# Autodesk Inventor assembly: 5_left_Arm
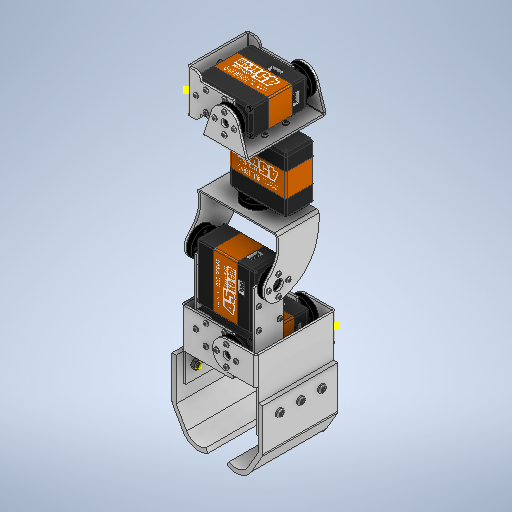
[picture p0: Inventor's stored thumbnail of the model, 512x512]
Saved by Autodesk Inventor 2026.1 (Build 301233000, 233)
## iProperties
Created: 2025-08-13
Part Number: 5_left_Arm
Document SubType Name: Assembly
Designer: LG
Author: LG
## Documents named in this file (18)
- C:\Users\LG\Desktop\RHp_Humanoid_ver1\Assembly\5_left_Arm.iam
- C:\Users\LG\Desktop\RHp_Humanoid_ver1\Part\HTD-45H, Horn\HTD-45H\HTD-45H.iam
- C:\Users\LG\Desktop\RHp_Humanoid_ver1\Part\HTD-45H, Horn\Horn\Top Horn.ipt
- C:\Users\LG\Desktop\RHp_Humanoid_ver1\Part\Frame\Arm\axis_13_top_frame.ipt
- C:\Users\LG\Desktop\RHp_Humanoid_ver1\Part\HTD-45H, Horn\Horn\Bottom Horn.ipt
- C:\Users\LG\Desktop\RHp_Humanoid_ver1\Part\Frame\Arm\axis_14_bottom_frame.ipt
- C:\Users\LG\Desktop\RHp_Humanoid_ver1\Part\Frame\Arm\HTD-45H_no bottom horn.ipt
- C:\Users\LG\Desktop\RHp_Humanoid_ver1\Part\Frame\Arm\axis_15_bottom_frame.ipt
- C:\Users\LG\Desktop\RHp_Humanoid_ver1\Part\Frame\Arm\axis_16_top_frame.ipt
- C:\Users\LG\Desktop\RHp_Humanoid_ver1\Part\Frame\Arm\axis_16_bottom_frame.ipt
- C:\Users\LG\Desktop\RHp_Humanoid_ver1\Part\Frame\Arm\axis_17_bottom_frame.ipt
- C:\Users\LG\Desktop\RHp_Humanoid_ver1\Part\Frame\Arm\axis_17_top_frame.ipt
- C:\Users\LG\Desktop\RHp_Humanoid_ver1\Part\Frame\Arm\gripper_frame.ipt
- C:\Users\LG\Desktop\RHp_Humanoid_ver1\Part\Bolt, Bearing, Nut, Washer\볼트, 너트\M2x4 Bolt.ipt
- C:\Users\LG\Desktop\RHp_Humanoid_ver1\Part\Bolt, Bearing, Nut, Washer\볼트, 너트\M2x6 Bolt.ipt
- C:\Users\LG\Desktop\RHp_Humanoid_ver1\Part\Bolt, Bearing, Nut, Washer\볼트, 너트\M3x6 Bolt.ipt
- C:\Users\LG\Desktop\RHp_Humanoid_ver1\Part\Bolt, Bearing, Nut, Washer\볼트, 너트\M3 Nut.ipt
- C:\Users\LG\Desktop\RHp_Humanoid_ver1\Part\Bolt, Bearing, Nut, Washer\볼트, 너트\M3x8 Bolt.ipt
## Components (104 placed, 16 different names)
1. M2x4 Bolt:51 — Rigid:82
2. M2x4 Bolt:54 — Rigid:84
3. M2x4 Bolt:53 — Rigid:83
4. M2x4 Bolt:52 — Rigid:85
5. M2x4 Bolt:3 — Rigid:5
6. M2x4 Bolt:2 — Rigid:7
7. M2x4 Bolt:4 — Rigid:6
8. M2x4 Bolt:1 — Rigid:3
9. M2x4 Bolt:5 — Rigid:4
10. M2x4 Bolt:8 — Rigid:8
11. M2x4 Bolt:6 — Rigid:10
12. M2x4 Bolt:9 — Rigid:11
13. M2x4 Bolt:7 — Rigid:9
14. Top Horn:1 — Mate:2, Mate:3, Mate:4
15. axis_13_top_frame:1 — Mate:2, Mate:3, Mate:4, Mate:5, Mate:6, Mate:7, Rigid:3, Rigid:4, Rigid:5, Rigid:6, Rigid:7, Rigid:8, Rigid:9, Rigid:10, Rigid:11, Rigid:82, Rigid:83, Rigid:84, Rigid:85
16. M2x4 Bolt:16 — Rigid:16
17. M2x4 Bolt:17 — Rigid:19
18. M2x4 Bolt:14 — Rigid:17
19. M2x4 Bolt:15 — Rigid:18
20. M2x4 Bolt:12 — Rigid:12
21. M2x4 Bolt:13 — Rigid:14
22. M2x4 Bolt:10 — Rigid:13
23. M2x4 Bolt:11 — Rigid:15
24. M2x4 Bolt:21 — Rigid:22
25. M2x4 Bolt:20 — Rigid:23
26. M2x4 Bolt:18 — Rigid:20
27. M2x4 Bolt:19 — Rigid:21
28. axis_14_bottom_frame:1 — Mate:10, Mate:11, Mate:12, Mate:13, Mate:14, Flush:4, Rigid:12, Rigid:13, Rigid:14, Rigid:15, Rigid:16, Rigid:17, Rigid:18, Rigid:19, Rigid:20, Rigid:21, Rigid:22, Rigid:23
29. Top Horn:2 — Rotational:2, Mate:10, Mate:11, Mate:12
30. Bottom Horn:1 — Mate:8, Mate:9, Flush:3
31. HTD-45H:2 [sub-assembly] — Mate:5, Mate:6, Mate:7, Rotational:2, Mate:8, Mate:9, Flush:3
32. M2x4 Bolt:25 — Rigid:24
33. M2x4 Bolt:24 — Rigid:27
34. M2x4 Bolt:23 — Rigid:26
35. M2x4 Bolt:22 — Rigid:25
36. M2x4 Bolt:30 — Rigid:32
37. M2x4 Bolt:32 — Rigid:33
38. M2x4 Bolt:31 — Rigid:34
39. M2x4 Bolt:33 — Rigid:35
40. M2x4 Bolt:26 — Rigid:28
41. M2x4 Bolt:28 — Rigid:30
42. M2x4 Bolt:27 — Rigid:29
43. M2x4 Bolt:29 — Rigid:31
44. axis_15_bottom_frame:1 — Mate:20, Mate:21, Mate:22, Mate:26, Mate:27, Mate:28, Rigid:24, Rigid:25, Rigid:26, Rigid:27, Rigid:28, Rigid:29, Rigid:30, Rigid:31, Rigid:32, Rigid:33, Rigid:34, Rigid:35
45. Top Horn:3 — Rotational:3, Mate:20, Mate:21, Mate:22
46. HTD-45H:3 — Mate:13, Mate:14, Flush:4, Rotational:3
47. M2x4 Bolt:34 — Rigid:36
48. M2x4 Bolt:35 — Rigid:38
49. M2x4 Bolt:36 — Rigid:37
50. M2x4 Bolt:37 — Rigid:39
51. M2x4 Bolt:42 — Rigid:40
52. M2x4 Bolt:40 — Rigid:42
53. M2x4 Bolt:38 — Rigid:41
54. M2x4 Bolt:39 — Rigid:43
55. M2x4 Bolt:41 — Rigid:86
56. M3x6 Bolt:3 — Rigid:64
57. M3x6 Bolt:2 — Rigid:65
58. M3x6 Bolt:4 — Rigid:62
59. M3x6 Bolt:1 — Rigid:63
60. M3 Nut:1 — Rigid:69
61. M3 Nut:4 — Rigid:67
62. M3 Nut:3 — Rigid:68
63. M3 Nut:2 — Rigid:66
64. axis_16_top_frame:1 — Mate:32, Mate:33, Mate:35, Mate:36, Mate:43, Rigid:36, Rigid:37, Rigid:38, Rigid:39, Rigid:40, Rigid:41, Rigid:42, Rigid:43, Rigid:62, Rigid:63, Rigid:64, Rigid:65, Rigid:86
65. axis_16_bottom_frame:1 — Mate:36, Mate:37, Flush:9, Mate:42, Flush:12, Rigid:66, Rigid:67, Rigid:68, Rigid:69
66. Top Horn:4 — Mate:26, Mate:27, Mate:28, Rotational:4
67. Bottom Horn:2 — Mate:29, Mate:30, Flush:6
68. HTD-45H:4 [sub-assembly] — Mate:29, Mate:30, Flush:6, Rotational:4, Mate:32, Mate:33, Mate:34, Flush:7, Flush:8
69. M2x4 Bolt:45 — Rigid:54
70. M2x4 Bolt:46 — Rigid:56
71. M2x4 Bolt:43 — Rigid:55
72. M2x4 Bolt:44 — Rigid:57
73. M2x4 Bolt:50 — Rigid:58
74. M2x4 Bolt:47 — Rigid:59
75. M2x4 Bolt:48 — Rigid:60
76. M2x4 Bolt:49 — Rigid:61
77. M2x6 Bolt:8 — Rigid:52
78. M2x6 Bolt:6 — Rigid:50
79. M2x6 Bolt:9 — Rigid:53
80. M2x6 Bolt:7 — Rigid:51
81. M2x6 Bolt:3 — Rigid:45
82. M2x6 Bolt:1 — Rigid:47
83. M2x6 Bolt:4 — Rigid:48
84. M2x6 Bolt:5 — Rigid:46
85. M2x6 Bolt:2 — Rigid:49
86. M3x8 Bolt:2 — Rigid:72
87. M3x8 Bolt:1 — Rigid:71
88. M3x8 Bolt:3 — Rigid:70
89. M3 Nut:5 — Rigid:73
90. M3 Nut:7 — Rigid:74
91. M3 Nut:6 — Rigid:75
92. M3x8 Bolt:4 — Rigid:76
93. M3x8 Bolt:5 — Rigid:77
94. M3x8 Bolt:6 — Rigid:78
95. M3 Nut:8 — Rigid:81
96. M3 Nut:9 — Rigid:80
97. M3 Nut:10 — Rigid:79
98. gripper_frame:2 — Rigid:2, Rigid:76, Rigid:77, Rigid:78
99. gripper_frame:1 — Rigid:1, Rigid:70, Rigid:71, Rigid:72
100. axis_17_bottom_frame:1 — Mate:40, Mate:41, Flush:11, Rigid:2, Rigid:54, Rigid:55, Rigid:56, Rigid:57, Rigid:58, Rigid:59, Rigid:60, Rigid:61, Rigid:79, Rigid:80, Rigid:81
101. axis_17_top_frame:1 — Mate:42, Flush:12, Mate:43, Rigid:1, Rigid:45, Rigid:46, Rigid:47, Rigid:48, Rigid:49, Rigid:50, Rigid:51, Rigid:52, Rigid:53, Rigid:73, Rigid:74, Rigid:75
102. Bottom Horn:3 — Mate:38, Mate:39, Flush:10
103. Top Horn:5 — Rotational:5, Mate:40, Mate:41, Flush:11
104. HTD-45H:5 [sub-assembly] — Mate:34, Flush:7, Flush:8, Mate:35, Mate:37, Flush:9, Rotational:5, Mate:38, Mate:39, Flush:10
## Relationships (131: WeldJoint 85, Mate 33, Flush 9, RevoluteJoint 4)
- Rotational:2 [RevoluteJoint]: Top Horn:2 ↔ HTD-45H:2
- Rotational:3 [RevoluteJoint]: Top Horn:3 ↔ HTD-45H:3
- Rotational:4 [RevoluteJoint]: Top Horn:4 ↔ HTD-45H:4
- Rotational:5 [RevoluteJoint]: Top Horn:5 ↔ HTD-45H:5
- Mate:2: Top Horn:1 ↔ axis_13_top_frame:1
- Mate:3: Top Horn:1 ↔ axis_13_top_frame:1
- Mate:4: Top Horn:1 ↔ axis_13_top_frame:1
- Mate:5: axis_13_top_frame:1 ↔ HTD-45H:2
- Mate:6: axis_13_top_frame:1 ↔ HTD-45H:2
- Mate:7 (2.5 mm): axis_13_top_frame:1 ↔ HTD-45H:2
- Mate:8: Bottom Horn:1 ↔ HTD-45H:2
- Mate:9: Bottom Horn:1 ↔ HTD-45H:2
- Flush:3: Bottom Horn:1 ↔ HTD-45H:2
- Mate:10: axis_14_bottom_frame:1 ↔ Top Horn:2
- Mate:11: axis_14_bottom_frame:1 ↔ Top Horn:2
- Mate:12 (14.5 mm): axis_14_bottom_frame:1 ↔ Top Horn:2
- Mate:13: axis_14_bottom_frame:1 ↔ HTD-45H:3
- Mate:14: axis_14_bottom_frame:1 ↔ HTD-45H:3
- Flush:4: axis_14_bottom_frame:1 ↔ HTD-45H:3
- Mate:20: axis_15_bottom_frame:1 ↔ Top Horn:3
- Mate:21: axis_15_bottom_frame:1 ↔ Top Horn:3
- Mate:22: axis_15_bottom_frame:1 ↔ Top Horn:3
- Mate:26: axis_15_bottom_frame:1 ↔ Top Horn:4
- Mate:27 (30.43 mm): axis_15_bottom_frame:1 ↔ Top Horn:4
- Mate:28 (-14 mm): axis_15_bottom_frame:1 ↔ Top Horn:4
- Mate:29: Bottom Horn:2 ↔ HTD-45H:4
- Mate:30: Bottom Horn:2 ↔ HTD-45H:4
- Flush:6: Bottom Horn:2 ↔ HTD-45H:4
- Mate:32: axis_16_top_frame:1 ↔ HTD-45H:4
- Mate:33: axis_16_top_frame:1 ↔ HTD-45H:4
- Mate:34 (3 mm): HTD-45H:4 ↔ HTD-45H:5
- Flush:7: HTD-45H:4 ↔ HTD-45H:5
- Flush:8: HTD-45H:4 ↔ HTD-45H:5
- Mate:35 (5 mm): axis_16_top_frame:1 ↔ HTD-45H:5
- Mate:36: axis_16_top_frame:1 ↔ axis_16_bottom_frame:1
- Mate:37: axis_16_bottom_frame:1 ↔ HTD-45H:5
- Flush:9: axis_16_bottom_frame:1 ↔ HTD-45H:5
- Mate:38: Bottom Horn:3 ↔ HTD-45H:5
- Mate:39: Bottom Horn:3 ↔ HTD-45H:5
- Flush:10: Bottom Horn:3 ↔ HTD-45H:5
- Mate:40: axis_17_bottom_frame:1 ↔ Top Horn:5
- Mate:41: axis_17_bottom_frame:1 ↔ Top Horn:5
- Flush:11 (19.43 mm): axis_17_bottom_frame:1 ↔ Top Horn:5
- Mate:42: axis_16_bottom_frame:1 ↔ axis_17_top_frame:1
- Flush:12: axis_16_bottom_frame:1 ↔ axis_17_top_frame:1
- Mate:43 (5 mm): axis_16_top_frame:1 ↔ axis_17_top_frame:1
- Rigid:1 [WeldJoint]: gripper_frame:1 ↔ axis_17_top_frame:1
- Rigid:2 [WeldJoint]: gripper_frame:2 ↔ axis_17_bottom_frame:1
- Rigid:3 [WeldJoint]: M2x4 Bolt:1 ↔ axis_13_top_frame:1
- Rigid:4 [WeldJoint]: M2x4 Bolt:5 ↔ axis_13_top_frame:1
- Rigid:5 [WeldJoint]: M2x4 Bolt:3 ↔ axis_13_top_frame:1
- Rigid:6 [WeldJoint]: M2x4 Bolt:4 ↔ axis_13_top_frame:1
- Rigid:7 [WeldJoint]: M2x4 Bolt:2 ↔ axis_13_top_frame:1
- Rigid:8 [WeldJoint]: M2x4 Bolt:8 ↔ axis_13_top_frame:1
- Rigid:9 [WeldJoint]: M2x4 Bolt:7 ↔ axis_13_top_frame:1
- Rigid:10 [WeldJoint]: M2x4 Bolt:6 ↔ axis_13_top_frame:1
- Rigid:11 [WeldJoint]: M2x4 Bolt:9 ↔ axis_13_top_frame:1
- Rigid:12 [WeldJoint]: M2x4 Bolt:12 ↔ axis_14_bottom_frame:1
- Rigid:13 [WeldJoint]: M2x4 Bolt:10 ↔ axis_14_bottom_frame:1
- Rigid:14 [WeldJoint]: M2x4 Bolt:13 ↔ axis_14_bottom_frame:1
- Rigid:15 [WeldJoint]: M2x4 Bolt:11 ↔ axis_14_bottom_frame:1
- Rigid:16 [WeldJoint]: M2x4 Bolt:16 ↔ axis_14_bottom_frame:1
- Rigid:17 [WeldJoint]: M2x4 Bolt:14 ↔ axis_14_bottom_frame:1
- Rigid:18 [WeldJoint]: M2x4 Bolt:15 ↔ axis_14_bottom_frame:1
- Rigid:19 [WeldJoint]: M2x4 Bolt:17 ↔ axis_14_bottom_frame:1
- Rigid:20 [WeldJoint]: M2x4 Bolt:18 ↔ axis_14_bottom_frame:1
- Rigid:21 [WeldJoint]: M2x4 Bolt:19 ↔ axis_14_bottom_frame:1
- Rigid:22 [WeldJoint]: M2x4 Bolt:21 ↔ axis_14_bottom_frame:1
- Rigid:23 [WeldJoint]: M2x4 Bolt:20 ↔ axis_14_bottom_frame:1
- Rigid:24 [WeldJoint]: M2x4 Bolt:25 ↔ axis_15_bottom_frame:1
- Rigid:25 [WeldJoint]: M2x4 Bolt:22 ↔ axis_15_bottom_frame:1
- Rigid:26 [WeldJoint]: M2x4 Bolt:23 ↔ axis_15_bottom_frame:1
- Rigid:27 [WeldJoint]: M2x4 Bolt:24 ↔ axis_15_bottom_frame:1
- Rigid:28 [WeldJoint]: M2x4 Bolt:26 ↔ axis_15_bottom_frame:1
- Rigid:29 [WeldJoint]: M2x4 Bolt:27 ↔ axis_15_bottom_frame:1
- Rigid:30 [WeldJoint]: M2x4 Bolt:28 ↔ axis_15_bottom_frame:1
- Rigid:31 [WeldJoint]: M2x4 Bolt:29 ↔ axis_15_bottom_frame:1
- Rigid:32 [WeldJoint]: M2x4 Bolt:30 ↔ axis_15_bottom_frame:1
- Rigid:33 [WeldJoint]: M2x4 Bolt:32 ↔ axis_15_bottom_frame:1
- Rigid:34 [WeldJoint]: M2x4 Bolt:31 ↔ axis_15_bottom_frame:1
- Rigid:35 [WeldJoint]: M2x4 Bolt:33 ↔ axis_15_bottom_frame:1
- Rigid:36 [WeldJoint]: M2x4 Bolt:34 ↔ axis_16_top_frame:1
- Rigid:37 [WeldJoint]: M2x4 Bolt:36 ↔ axis_16_top_frame:1
- Rigid:38 [WeldJoint]: M2x4 Bolt:35 ↔ axis_16_top_frame:1
- Rigid:39 [WeldJoint]: M2x4 Bolt:37 ↔ axis_16_top_frame:1
- Rigid:40 [WeldJoint]: M2x4 Bolt:42 ↔ axis_16_top_frame:1
- Rigid:41 [WeldJoint]: M2x4 Bolt:38 ↔ axis_16_top_frame:1
- Rigid:42 [WeldJoint]: M2x4 Bolt:40 ↔ axis_16_top_frame:1
- Rigid:43 [WeldJoint]: M2x4 Bolt:39 ↔ axis_16_top_frame:1
- Rigid:45 [WeldJoint]: M2x6 Bolt:3 ↔ axis_17_top_frame:1
- Rigid:46 [WeldJoint]: M2x6 Bolt:5 ↔ axis_17_top_frame:1
- Rigid:47 [WeldJoint]: M2x6 Bolt:1 ↔ axis_17_top_frame:1
- Rigid:48 [WeldJoint]: M2x6 Bolt:4 ↔ axis_17_top_frame:1
- Rigid:49 [WeldJoint]: M2x6 Bolt:2 ↔ axis_17_top_frame:1
- Rigid:50 [WeldJoint]: M2x6 Bolt:6 ↔ axis_17_top_frame:1
- Rigid:51 [WeldJoint]: M2x6 Bolt:7 ↔ axis_17_top_frame:1
- Rigid:52 [WeldJoint]: M2x6 Bolt:8 ↔ axis_17_top_frame:1
- Rigid:53 [WeldJoint]: M2x6 Bolt:9 ↔ axis_17_top_frame:1
- Rigid:54 [WeldJoint]: M2x4 Bolt:45 ↔ axis_17_bottom_frame:1
- Rigid:55 [WeldJoint]: M2x4 Bolt:43 ↔ axis_17_bottom_frame:1
- Rigid:56 [WeldJoint]: M2x4 Bolt:46 ↔ axis_17_bottom_frame:1
- Rigid:57 [WeldJoint]: M2x4 Bolt:44 ↔ axis_17_bottom_frame:1
- Rigid:58 [WeldJoint]: M2x4 Bolt:50 ↔ axis_17_bottom_frame:1
- Rigid:59 [WeldJoint]: M2x4 Bolt:47 ↔ axis_17_bottom_frame:1
- Rigid:60 [WeldJoint]: M2x4 Bolt:48 ↔ axis_17_bottom_frame:1
- Rigid:61 [WeldJoint]: M2x4 Bolt:49 ↔ axis_17_bottom_frame:1
- Rigid:62 [WeldJoint]: M3x6 Bolt:4 ↔ axis_16_top_frame:1
- Rigid:63 [WeldJoint]: M3x6 Bolt:1 ↔ axis_16_top_frame:1
- Rigid:64 [WeldJoint]: M3x6 Bolt:3 ↔ axis_16_top_frame:1
- Rigid:65 [WeldJoint]: M3x6 Bolt:2 ↔ axis_16_top_frame:1
- Rigid:66 [WeldJoint]: M3 Nut:2 ↔ axis_16_bottom_frame:1
- Rigid:67 [WeldJoint]: M3 Nut:4 ↔ axis_16_bottom_frame:1
- Rigid:68 [WeldJoint]: M3 Nut:3 ↔ axis_16_bottom_frame:1
- Rigid:69 [WeldJoint]: M3 Nut:1 ↔ axis_16_bottom_frame:1
- Rigid:70 [WeldJoint]: M3x8 Bolt:3 ↔ gripper_frame:1
- Rigid:71 [WeldJoint]: M3x8 Bolt:1 ↔ gripper_frame:1
- Rigid:72 [WeldJoint]: M3x8 Bolt:2 ↔ gripper_frame:1
- Rigid:73 [WeldJoint]: M3 Nut:5 ↔ axis_17_top_frame:1
- Rigid:74 [WeldJoint]: M3 Nut:7 ↔ axis_17_top_frame:1
- Rigid:75 [WeldJoint]: M3 Nut:6 ↔ axis_17_top_frame:1
- Rigid:76 [WeldJoint]: M3x8 Bolt:4 ↔ gripper_frame:2
- Rigid:77 [WeldJoint]: M3x8 Bolt:5 ↔ gripper_frame:2
- Rigid:78 [WeldJoint]: M3x8 Bolt:6 ↔ gripper_frame:2
- Rigid:79 [WeldJoint]: M3 Nut:10 ↔ axis_17_bottom_frame:1
- Rigid:80 [WeldJoint]: M3 Nut:9 ↔ axis_17_bottom_frame:1
- Rigid:81 [WeldJoint]: M3 Nut:8 ↔ axis_17_bottom_frame:1
- Rigid:82 [WeldJoint]: M2x4 Bolt:51 ↔ axis_13_top_frame:1
- Rigid:83 [WeldJoint]: M2x4 Bolt:53 ↔ axis_13_top_frame:1
- Rigid:84 [WeldJoint]: M2x4 Bolt:54 ↔ axis_13_top_frame:1
- Rigid:85 [WeldJoint]: M2x4 Bolt:52 ↔ axis_13_top_frame:1
- Rigid:86 [WeldJoint]: M2x4 Bolt:41 ↔ axis_16_top_frame:1
